# Autodesk Inventor assembly: Roller-ver2-1111-2021
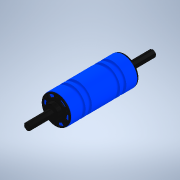
[picture p0: Inventor's stored thumbnail of the model, 180x180]
Saved by Autodesk Inventor 2021 (Build 250183000, 183)
## iProperties
Created: 2021-03-22
Part Number: Roller-ver2-1111-2021
Document SubType Name: Assembly
Designer: CMurray
Author: CMurray
## Documents named in this file (4)
- C:\Users\CMurray\OneDrive\Documents\GitHub\RoboticsCad1111\PHRC CADD\2020 Infinite Recharge\Storage\Assemblies\Roller-ver2-1111-2021.iam
- F:\PHRC CADD 2021\PHRC CADD\2020 Infinite Recharge\Storage\Parts\Roller-ver3-1111-2019.ipt
- F:\PHRC CADD 2021\PHRC CADD\Resources\VEXpro Resources\Versa Motion\VersaHub(0.5inHex)-1111-2016.ipt
- F:\PHRC CADD 2021\PHRC CADD\Resources\VEXpro Resources\Shafts\0.5inThunderHexShaft(18in)-1111-2016.ipt
## Components (4 placed, 3 different names)
1. Roller-ver3-1111-2019:1 — Cylindrical:1, Flush:1, Mate:2, Mate:3
2. 0.5inThunderHexShaft(18in)-1111-2016:1 — Cylindrical:1, Mate:1, Angle:1, Flush:1, Cylindrical:2, Angle:2, Cylindrical:3
3. VersaHub(0.5inHex)-1111-2016:1 — Cylindrical:2, Mate:2, Angle:2
4. VersaHub(0.5inHex)-1111-2016:2 — Cylindrical:3, Mate:3
## Relationships (9: CylindricalJoint 3, Mate 3, Angle 2, Flush 1)
- Cylindrical:1: Roller-ver3-1111-2019:1 ↔ 0.5inThunderHexShaft(18in)-1111-2016:1
- Mate:1: 0.5inThunderHexShaft(18in)-1111-2016:1
- Angle:1 (0 deg): 0.5inThunderHexShaft(18in)-1111-2016:1
- Flush:1 (-60.325 mm): Roller-ver3-1111-2019:1 ↔ 0.5inThunderHexShaft(18in)-1111-2016:1
- Cylindrical:2: 0.5inThunderHexShaft(18in)-1111-2016:1 ↔ VersaHub(0.5inHex)-1111-2016:1
- Mate:2: Roller-ver3-1111-2019:1 ↔ VersaHub(0.5inHex)-1111-2016:1
- Angle:2 (90 deg): 0.5inThunderHexShaft(18in)-1111-2016:1 ↔ VersaHub(0.5inHex)-1111-2016:1
- Cylindrical:3: 0.5inThunderHexShaft(18in)-1111-2016:1 ↔ VersaHub(0.5inHex)-1111-2016:2
- Mate:3: Roller-ver3-1111-2019:1 ↔ VersaHub(0.5inHex)-1111-2016:2
